# Autodesk Inventor assembly: gopro_assembly
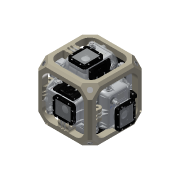
[picture p0: Inventor's stored thumbnail of the model, 180x180]
Saved by Autodesk Inventor 2015 (Build 190159000, 159)
## iProperties
Created: 2014-07-12
Part Number: gopro_assembly
Document SubType Name: Assembly
Designer: Antonella Wilby
Author: Antonella Wilby
## Documents named in this file (4)
- C:\Users\Antonella\Documents\Inventor\GoProCube\gopro_360_external.iam
- C:\Users\Antonella\Documents\Inventor\GoProCube\gopro_360_external.ipt
- C:\Users\Antonella\Documents\Inventor\GoProCube\GoPro Hero 3 White\GoPro_Hero_3_White.iam
- C:\Users\Antonella\Documents\Inventor\GoProCube\threaded_insert_1-4-20.ipt
## Components (15 placed, 3 different names)
1. gopro_360_external:1 — Mate:1, Mate:2, Angle:1, Mate:3, Mate:4, Angle:2, Mate:5, Mate:6, Angle:3, Mate:7, Mate:8, Angle:4, Mate:9, Mate:10, Angle:5, Mate:11, Mate:12, Angle:6, Mate:13, Mate:14, Mate:15, Mate:16, Mate:17, Mate:18, Mate:19, Mate:20, Mate:21, Mate:22, Mate:23, Mate:24, Mate:25, Mate:26, Mate:27, Mate:28
2. GoPro_Hero_3_White:1 [sub-assembly] — Mate:1, Mate:2, Angle:1
3. GoPro_Hero_3_White:2 [sub-assembly] — Mate:3, Mate:4, Angle:2
4. GoPro_Hero_3_White:3 [sub-assembly] — Mate:5, Mate:6, Angle:3
5. GoPro_Hero_3_White:4 [sub-assembly] — Mate:7, Mate:8, Angle:4
6. GoPro_Hero_3_White:5 [sub-assembly] — Mate:9, Mate:10, Angle:5
7. GoPro_Hero_3_White:6 [sub-assembly] — Mate:11, Mate:12, Angle:6
8. threaded_insert_1-4-20:1 — Mate:13, Mate:14
9. threaded_insert_1-4-20:2 — Mate:15, Mate:16
10. threaded_insert_1-4-20:3 — Mate:17, Mate:18
11. threaded_insert_1-4-20:4 — Mate:19, Mate:20
12. threaded_insert_1-4-20:5 — Mate:21, Mate:22
13. threaded_insert_1-4-20:6 — Mate:23, Mate:24
14. threaded_insert_1-4-20:7 — Mate:25, Mate:26
15. threaded_insert_1-4-20:8 — Mate:27, Mate:28
## Relationships (34: Mate 28, Angle 6)
- Mate:1: gopro_360_external:1 ↔ GoPro_Hero_3_White:1
- Mate:2: gopro_360_external:1 ↔ GoPro_Hero_3_White:1
- Angle:1 (0 deg): gopro_360_external:1 ↔ GoPro_Hero_3_White:1
- Mate:3: gopro_360_external:1 ↔ GoPro_Hero_3_White:2
- Mate:4: gopro_360_external:1 ↔ GoPro_Hero_3_White:2
- Angle:2 (0 deg): gopro_360_external:1 ↔ GoPro_Hero_3_White:2
- Mate:5: gopro_360_external:1 ↔ GoPro_Hero_3_White:3
- Mate:6: gopro_360_external:1 ↔ GoPro_Hero_3_White:3
- Angle:3 (0 deg): gopro_360_external:1 ↔ GoPro_Hero_3_White:3
- Mate:7: gopro_360_external:1 ↔ GoPro_Hero_3_White:4
- Mate:8: gopro_360_external:1 ↔ GoPro_Hero_3_White:4
- Angle:4 (0 deg): gopro_360_external:1 ↔ GoPro_Hero_3_White:4
- Mate:9: gopro_360_external:1 ↔ GoPro_Hero_3_White:5
- Mate:10: gopro_360_external:1 ↔ GoPro_Hero_3_White:5
- Angle:5 (0 deg): gopro_360_external:1 ↔ GoPro_Hero_3_White:5
- Mate:11: gopro_360_external:1 ↔ GoPro_Hero_3_White:6
- Mate:12: gopro_360_external:1 ↔ GoPro_Hero_3_White:6
- Angle:6 (0 deg): gopro_360_external:1 ↔ GoPro_Hero_3_White:6
- Mate:13: gopro_360_external:1 ↔ threaded_insert_1-4-20:1
- Mate:14: gopro_360_external:1 ↔ threaded_insert_1-4-20:1
- Mate:15: gopro_360_external:1 ↔ threaded_insert_1-4-20:2
- Mate:16: gopro_360_external:1 ↔ threaded_insert_1-4-20:2
- Mate:17: gopro_360_external:1 ↔ threaded_insert_1-4-20:3
- Mate:18: gopro_360_external:1 ↔ threaded_insert_1-4-20:3
- Mate:19: gopro_360_external:1 ↔ threaded_insert_1-4-20:4
- Mate:20: gopro_360_external:1 ↔ threaded_insert_1-4-20:4
- Mate:21: gopro_360_external:1 ↔ threaded_insert_1-4-20:5
- Mate:22: gopro_360_external:1 ↔ threaded_insert_1-4-20:5
- Mate:23: gopro_360_external:1 ↔ threaded_insert_1-4-20:6
- Mate:24: gopro_360_external:1 ↔ threaded_insert_1-4-20:6
- Mate:25: gopro_360_external:1 ↔ threaded_insert_1-4-20:7
- Mate:26: gopro_360_external:1 ↔ threaded_insert_1-4-20:7
- Mate:27: gopro_360_external:1 ↔ threaded_insert_1-4-20:8
- Mate:28: gopro_360_external:1 ↔ threaded_insert_1-4-20:8
